# Autodesk Inventor assembly: ServoBlockLargeServoPlateWithStandoffs
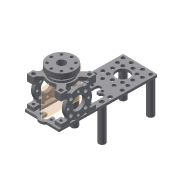
[picture p0: Inventor's stored thumbnail of the model, 180x180]
Saved by Autodesk Inventor 2018 (Build 220112000, 112)
## iProperties
Created: 2018-10-26
Part Number: ServoBlockLargeServoPlateWithStandoffs
Document SubType Name: Assembly
Designer: ball
Author: ball
## Documents named in this file (3)
- C:\FTC\FTC8863CAD\2018Robot\ServoBlockLargeServoPlateWithStandoffs.iam
- C:\FTC\FTC8863CAD\2018Robot\ServoBlockLargeServoPlate.iam
- C:\FTC\FTC8863CAD\Actobotics\633 parts\633134.ipt
## Components (5 placed, 2 different names)
1. ServoBlockLargeServoPlate:1 [sub-assembly] — Mate:1, Mate:2, Mate:3, Mate:4, Mate:5, Mate:6, Mate:7, Mate:8
2. 633134:1 — Mate:2, Mate:7
3. 633134:2 — Mate:1, Mate:6
4. 633134:3 — Mate:4, Mate:8
5. 633134:4 — Mate:3, Mate:5
## Relationships (8: Mate 8)
- Mate:1: ServoBlockLargeServoPlate:1 ↔ 633134:2
- Mate:2: ServoBlockLargeServoPlate:1 ↔ 633134:1
- Mate:3: ServoBlockLargeServoPlate:1 ↔ 633134:4
- Mate:4: ServoBlockLargeServoPlate:1 ↔ 633134:3
- Mate:5: ServoBlockLargeServoPlate:1 ↔ 633134:4
- Mate:6: ServoBlockLargeServoPlate:1 ↔ 633134:2
- Mate:7: ServoBlockLargeServoPlate:1 ↔ 633134:1
- Mate:8: ServoBlockLargeServoPlate:1 ↔ 633134:3
